# Autodesk Inventor assembly: WheelAssembly3.0
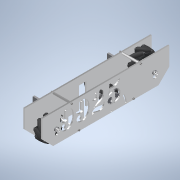
[picture p0: Inventor's stored thumbnail of the model, 180x180]
Saved by Autodesk Inventor 2021 (Build 250183000, 183)
## iProperties
Created: 2017-07-22
Part Number: WheelAssembly3.0
Document SubType Name: Assembly
Designer: User
Mass: 2301.48 g
Surface Area: 4071.67 cm^2
Volume: 902.346 cm^3
Density: 2.55055 g/cm^3
Author: User
## Documents named in this file (21)
- D:\robotics\CAD\2020-21-CAD\Drivetrain\drive train right.iam
- D:\robotics\CAD\COTSParts\Actobotics\535 parts\535198Bearing.25ID.5OD.ipt
- D:\robotics\CAD\COTSParts\Actobotics\Collar.ipt
- D:\robotics\CAD\COTSParts\Fasteners\6-32 SHCS x500.ipt
- D:\robotics\CAD\COTSParts\Fasteners\Hex Standoff 6-32 x2250.ipt
- D:\robotics\CAD\2020-21-CAD\Drivetrain\motor mount_MIR.ipt
- D:\robotics\CAD\COTSParts\Rev\REV-41-1657MecanumWheelRight.iam
- D:\robotics\CAD\2020-21-CAD\Drivetrain\motor mount.ipt
- D:\robotics\CAD\COTSParts\Tetrix\Tetrix hub - motor.ipt
- D:\robotics\CAD\COTSParts\Actobotics\535 parts\535198Bearing.25ID.5OD_MIR1.ipt
- D:\robotics\CAD\COTSParts\Actobotics\Collar_MIR1.ipt
- D:\robotics\CAD\COTSParts\Rev\REV-41-1657MecanumWheelRight_MIR.iam
- D:\robotics\CAD\COTSParts\Motors\am-3102NeveRest20 (1)_MIR_MIR.ipt
- D:\robotics\CAD\COTSParts\andymark\am-3902 am-3903 2in Omni 14mm Hex.ipt
- D:\robotics\CAD\COTSParts\Rev\REV-11-1271.STEP encoders.ipt
- D:\robotics\CAD\COTSParts\Actobotics\637 parts\637222 beval gear\615456 13tooth beval gear.ipt
- D:\robotics\CAD\COTSParts\Actobotics\637 parts\637222 beval gear\615460 26 tooth beval gear.ipt
- D:\robotics\CAD\COTSParts\Tetrix\Tetrix Hub - axle.ipt
- D:\robotics\CAD\COTSParts\Motors\am-3102NeveRest20 (1).ipt
- D:\robotics\CAD\2020-21-CAD\Drivetrain\InvertedDrivePlateInsideright.ipt
- D:\robotics\CAD\2020-21-CAD\Drivetrain\InvertedDrivePlateOutsideright.ipt
## Components (35 placed, 20 different names)
1. 535198Bearing.25ID.5OD:1 — Insert:86
2. Collar:1 — Insert:86
3. 535198Bearing.25ID.5OD:5
4. Hex Standoff 6-32 x2250:1 — Mate:108, Mate:117, Mate:118
5. Hex Standoff 6-32 x2250:2 — Mate:106, Mate:107, Mate:110, Mate:111
6. Hex Standoff 6-32 x2250:3 — Mate:115, Mate:116
7. Hex Standoff 6-32 x2250:4 — Mate:109, Mate:112, Mate:114
8. 6-32 SHCS x500:22 — Mate:123, Mate:124
9. 6-32 SHCS x500:23 — Mate:138, Mate:139
10. 6-32 SHCS x500:24 — Mate:125, Mate:126, Mate:127
11. 6-32 SHCS x500:25 — Mate:121, Mate:122
12. 6-32 SHCS x500:26
13. 6-32 SHCS x500:27 — Mate:140, Mate:141
14. 6-32 SHCS x500:28 — Mate:119, Mate:120
15. 6-32 SHCS x500:29 — Mate:113
16. REV-41-1657MecanumWheelRight:1 [sub-assembly] — Mate:70, Mate:71, Mate:72, Flush:14, Mate:137
17. motor mount:1 — Mate:103, Flush:15, Flush:16, Flush:17, Mate:128, Mate:129, Mate:130
18. Tetrix hub - motor:1 — Mate:70, Mate:71, Mate:72, Mate:136
19. 535198Bearing.25ID.5OD_MIR1:1 — Insert:151
20. Collar_MIR1:1 — Insert:151
21. 535198Bearing.25ID.5OD_MIR1:2
22. REV-41-1657MecanumWheelRight_MIR:1 [sub-assembly] — Flush:14
23. motor mount_MIR:1 — Mate:78, Mate:79, Mate:95, Flush:16, Angle:4, Flush:17, Mate:131
24. am-3102NeveRest20 (1)_MIR_MIR:1 — Mate:78, Mate:79, Mate:96, Angle:4
25. am-3902 am-3903 2in Omni 14mm Hex:1 — Mate:89, Mate:90
26. REV-11-1271.STEP encoders:1 — Mate:89, Mate:90
27. 615456 13tooth beval gear:1 — Mate:105, Mate:132
28. 615460 26 tooth beval gear:1 — Mate:93, Mate:94, Mate:96, Mate:105
29. Tetrix Hub - axle:1 — Mate:93, Mate:94, Mate:95
30. 615460 26 tooth beval gear:2 — Mate:104, Mate:135
31. Tetrix Hub - axle:2
32. am-3102NeveRest20 (1):1 — Mate:103, Flush:15, Mate:104
33. InvertedDrivePlateInsideright:1 — Mate:110, Mate:111, Mate:113, Mate:114, Mate:115, Mate:117, Mate:119, Mate:120, Mate:128, Mate:129, Mate:130, Mate:131, Mate:132, Mate:133, Mate:134, Mate:140, Mate:141
34. InvertedDrivePlateOutsideright:1 — Mate:106, Mate:107, Mate:108, Mate:109, Mate:112, Mate:116, Mate:118, Mate:121, Mate:122, Mate:123, Mate:124, Mate:125, Mate:126, Mate:127, Mate:136, Mate:137, Mate:138, Mate:139
35. 615456 13tooth beval gear:2 — Mate:133, Mate:134, Mate:135
## Relationships (59: Mate 52, Flush 4, Insert 2, Angle 1)
- Insert:86: 535198Bearing.25ID.5OD:1 ↔ Collar:1
- Mate:70: REV-41-1657MecanumWheelRight:1 ↔ Tetrix hub - motor:1
- Mate:71: REV-41-1657MecanumWheelRight:1 ↔ Tetrix hub - motor:1
- Mate:72: REV-41-1657MecanumWheelRight:1 ↔ Tetrix hub - motor:1
- Insert:151: 535198Bearing.25ID.5OD_MIR1:1 ↔ Collar_MIR1:1
- Mate:78: motor mount_MIR:1 ↔ am-3102NeveRest20 (1)_MIR_MIR:1
- Mate:79: motor mount_MIR:1 ↔ am-3102NeveRest20 (1)_MIR_MIR:1
- Flush:14: REV-41-1657MecanumWheelRight:1 ↔ REV-41-1657MecanumWheelRight_MIR:1
- Mate:89: am-3902 am-3903 2in Omni 14mm Hex:1 ↔ REV-11-1271.STEP encoders:1
- Mate:90: am-3902 am-3903 2in Omni 14mm Hex:1 ↔ REV-11-1271.STEP encoders:1
- Mate:93: 615460 26 tooth beval gear:1 ↔ Tetrix Hub - axle:1
- Mate:94: 615460 26 tooth beval gear:1 ↔ Tetrix Hub - axle:1
- Mate:95 (19.05 mm): motor mount_MIR:1 ↔ Tetrix Hub - axle:1
- Mate:96: am-3102NeveRest20 (1)_MIR_MIR:1 ↔ 615460 26 tooth beval gear:1
- [Mate]: 615460 26 tooth beval gear:2 ↔ Tetrix Hub - axle:2
- [Mate]: 615460 26 tooth beval gear:2 ↔ Tetrix Hub - axle:2
- Mate:103: motor mount:1 ↔ am-3102NeveRest20 (1):1
- Flush:15: motor mount:1 ↔ am-3102NeveRest20 (1):1
- Mate:104: 615460 26 tooth beval gear:2 ↔ am-3102NeveRest20 (1):1
- Flush:16: motor mount:1 ↔ motor mount_MIR:1
- Angle:4 (17 deg): motor mount_MIR:1 ↔ am-3102NeveRest20 (1)_MIR_MIR:1
- Mate:105: 615456 13tooth beval gear:1 ↔ 615460 26 tooth beval gear:1
- Mate:106: Hex Standoff 6-32 x2250:2 ↔ InvertedDrivePlateOutsideright:1
- Mate:107: Hex Standoff 6-32 x2250:2 ↔ InvertedDrivePlateOutsideright:1
- Mate:108: Hex Standoff 6-32 x2250:1 ↔ InvertedDrivePlateOutsideright:1
- Mate:109: Hex Standoff 6-32 x2250:4 ↔ InvertedDrivePlateOutsideright:1
- Mate:110: Hex Standoff 6-32 x2250:2 ↔ InvertedDrivePlateInsideright:1
- Mate:111: Hex Standoff 6-32 x2250:2 ↔ InvertedDrivePlateInsideright:1
- Mate:112: Hex Standoff 6-32 x2250:4 ↔ InvertedDrivePlateOutsideright:1
- Mate:113: 6-32 SHCS x500:29 ↔ InvertedDrivePlateInsideright:1
- Mate:114: Hex Standoff 6-32 x2250:4 ↔ InvertedDrivePlateInsideright:1
- Mate:115: Hex Standoff 6-32 x2250:3 ↔ InvertedDrivePlateInsideright:1
- Mate:116: Hex Standoff 6-32 x2250:3 ↔ InvertedDrivePlateOutsideright:1
- Mate:117: Hex Standoff 6-32 x2250:1 ↔ InvertedDrivePlateInsideright:1
- Mate:118: Hex Standoff 6-32 x2250:1 ↔ InvertedDrivePlateOutsideright:1
- Mate:119: 6-32 SHCS x500:28 ↔ InvertedDrivePlateInsideright:1
- Mate:120: 6-32 SHCS x500:28 ↔ InvertedDrivePlateInsideright:1
- Mate:121: 6-32 SHCS x500:25 ↔ InvertedDrivePlateOutsideright:1
- Mate:122: 6-32 SHCS x500:25 ↔ InvertedDrivePlateOutsideright:1
- Mate:123: 6-32 SHCS x500:22 ↔ InvertedDrivePlateOutsideright:1
- Mate:124: 6-32 SHCS x500:22 ↔ InvertedDrivePlateOutsideright:1
- Mate:125: 6-32 SHCS x500:24 ↔ InvertedDrivePlateOutsideright:1
- Mate:126: 6-32 SHCS x500:24 ↔ InvertedDrivePlateOutsideright:1
- Mate:127: 6-32 SHCS x500:24 ↔ InvertedDrivePlateOutsideright:1
- Flush:17: motor mount:1 ↔ motor mount_MIR:1
- Mate:128: motor mount:1 ↔ InvertedDrivePlateInsideright:1
- Mate:129: motor mount:1 ↔ InvertedDrivePlateInsideright:1
- Mate:130: motor mount:1 ↔ InvertedDrivePlateInsideright:1
- Mate:131: motor mount_MIR:1 ↔ InvertedDrivePlateInsideright:1
- Mate:132: 615456 13tooth beval gear:1 ↔ InvertedDrivePlateInsideright:1
- Mate:133: InvertedDrivePlateInsideright:1 ↔ 615456 13tooth beval gear:2
- Mate:134: InvertedDrivePlateInsideright:1 ↔ 615456 13tooth beval gear:2
- Mate:135: 615460 26 tooth beval gear:2 ↔ 615456 13tooth beval gear:2
- Mate:136: Tetrix hub - motor:1 ↔ InvertedDrivePlateOutsideright:1
- Mate:137 (25.4 mm): REV-41-1657MecanumWheelRight:1 ↔ InvertedDrivePlateOutsideright:1
- Mate:138: 6-32 SHCS x500:23 ↔ InvertedDrivePlateOutsideright:1
- Mate:139: 6-32 SHCS x500:23 ↔ InvertedDrivePlateOutsideright:1
- Mate:140: 6-32 SHCS x500:27 ↔ InvertedDrivePlateInsideright:1
- Mate:141: 6-32 SHCS x500:27 ↔ InvertedDrivePlateInsideright:1
## Named parameters: d366_d360 = 0 mm, d367_d361 = 0 mm
